# Autodesk Inventor assembly: Moteur + laser
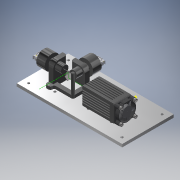
[picture p0: Inventor's stored thumbnail of the model, 180x180]
Saved by Autodesk Inventor 2017 (Build 210142000, 142)
## iProperties
Part Number: Moteur + laser
Material: Générique
Document SubType Name: Assembly
Designer: Adrien MARY
Stock Number: 1410-02-00
Project: 1410 LaserShow
Author: Adrien MARY
## Documents named in this file (9)
- W:\Professionnel\Conception FABLAB\1410-LaserShow\1410-02 Moteur + laser\1410-02-00 Moteur + Laser.iam
- W:\Professionnel\Conception FABLAB\1410-LaserShow\1410-02 Moteur + laser\1410-02 Plaque support.ipt
- W:\Professionnel\Conception FABLAB\1410-LaserShow\1410-03 Composant electronique\1410-03-09 Laser.ipt
- W:\Professionnel\Conception FABLAB\1410-LaserShow\1410-03 Composant electronique\1410-03-10 Moteur+mirroir.ipt
- W:\Professionnel\Conception FABLAB\1410-LaserShow\1410-90 Centre de contenu\fr-FR\ISO 4762(2)\ISO 4762 - M3 x 10ISO.ipt
- W:\Professionnel\Conception FABLAB\1410-LaserShow\1410-03 Composant electronique\1410-03-11 Ventilateur 30x30.ipt
- W:\Professionnel\Conception FABLAB\1410-LaserShow\1410-90 Centre de contenu\fr-FR\ISO 4762(2)\ISO 4762 - M3 x 12ISO.ipt
- W:\Professionnel\Conception FABLAB\1410-LaserShow\1410-90 Centre de contenu\fr-FR\ISO 4762(2)\ISO 4762 - M3 x 16ISO.ipt
- W:\Professionnel\Conception FABLAB\1410-LaserShow\1410-90 Centre de contenu\fr-FR\ISO 4032(2)\ISO 4032 - M3 - ISO.ipt
## Components (19 placed, 8 different names)
1. 1410-02 Plaque support:1 — Logement:12, Logement:13, Logement:14, Logement:15, Logement:16, Logement:17, Logement:18, Logement:19, Logement:20, Placage:3, Placage:4, Logement:25, Logement:26, Logement:27, Logement:28, Placage:5
2. 1410-03-09 Laser:1 — Placage:1, Placage:3, Placage:4, Placage:5, Placage:6, Placage:7
3. 1410-03-10 Moteur+mirroir:1 — Logement:12, Logement:13
4. ISO 4762 M3 x 10:1 — Logement:16
5. ISO 4762 M3 x 10:3 — Logement:14
6. ISO 4762 M3 x 10:2 — Logement:15
7. ISO 4762 M3 x 16:1 — Logement:20
8. ISO 4762 M3 x 16:2 — Logement:19
9. ISO 4762 M3 x 16:3 — Logement:17
10. ISO 4762 M3 x 16:4 — Logement:18
11. 1410-03-11 Ventilateur 30x30:1 — Placage:1, Logement:21, Logement:22, Logement:23, Logement:24
12. ISO 4762 M3 x 12:1 — Logement:21, Placage:7
13. ISO 4762 M3 x 12:2 — Logement:22
14. ISO 4762 M3 x 12:3 — Logement:23, Placage:6
15. ISO 4762 M3 x 12:4 — Logement:24
16. ISO 4032 M3:1 — Logement:28
17. ISO 4032 M3:2 — Logement:27
18. ISO 4032 M3:3 — Logement:25
19. ISO 4032 M3:4 — Logement:26
## Relationships (23: Insert 17, Mate 6)
- Logement:12 [Insert]: 1410-02 Plaque support:1 ↔ 1410-03-10 Moteur+mirroir:1
- Logement:13 [Insert]: 1410-02 Plaque support:1 ↔ 1410-03-10 Moteur+mirroir:1
- Logement:14 [Insert]: 1410-02 Plaque support:1 ↔ ISO 4762 M3 x 10:3
- Logement:15 [Insert]: 1410-02 Plaque support:1 ↔ ISO 4762 M3 x 10:2
- Logement:16 [Insert]: 1410-02 Plaque support:1 ↔ ISO 4762 M3 x 10:1
- Logement:17 [Insert]: 1410-02 Plaque support:1 ↔ ISO 4762 M3 x 16:3
- Logement:18 [Insert]: 1410-02 Plaque support:1 ↔ ISO 4762 M3 x 16:4
- Logement:19 [Insert]: 1410-02 Plaque support:1 ↔ ISO 4762 M3 x 16:2
- Logement:20 [Insert]: 1410-02 Plaque support:1 ↔ ISO 4762 M3 x 16:1
- Placage:1 [Mate]: 1410-03-09 Laser:1 ↔ 1410-03-11 Ventilateur 30x30:1
- Logement:21 [Insert]: 1410-03-11 Ventilateur 30x30:1 ↔ ISO 4762 M3 x 12:1
- Logement:22 [Insert]: 1410-03-11 Ventilateur 30x30:1 ↔ ISO 4762 M3 x 12:2
- Logement:23 [Insert]: 1410-03-11 Ventilateur 30x30:1 ↔ ISO 4762 M3 x 12:3
- Logement:24 [Insert]: 1410-03-11 Ventilateur 30x30:1 ↔ ISO 4762 M3 x 12:4
- Placage:3 [Mate]: 1410-02 Plaque support:1 ↔ 1410-03-09 Laser:1
- Placage:4 [Mate]: 1410-02 Plaque support:1 ↔ 1410-03-09 Laser:1
- Logement:25 [Insert]: 1410-02 Plaque support:1 ↔ ISO 4032 M3:3
- Logement:26 [Insert]: 1410-02 Plaque support:1 ↔ ISO 4032 M3:4
- Logement:27 [Insert]: 1410-02 Plaque support:1 ↔ ISO 4032 M3:2
- Logement:28 [Insert]: 1410-02 Plaque support:1 ↔ ISO 4032 M3:1
- Placage:5 [Mate] (5 mm): 1410-02 Plaque support:1 ↔ 1410-03-09 Laser:1
- Placage:6 [Mate]: 1410-03-09 Laser:1 ↔ ISO 4762 M3 x 12:3
- Placage:7 [Mate]: 1410-03-09 Laser:1 ↔ ISO 4762 M3 x 12:1
